# Autodesk Inventor assembly: Chimera Assembly
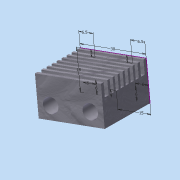
[picture p0: Inventor's stored thumbnail of the model, 180x180]
Saved by Autodesk Inventor 2016 (Build 200138000, 138)
## iProperties
Created: 2016-08-02
Part Number: Chimera Assembly
Document SubType Name: Assembly
Designer: Sam
Author: Sam
## Documents named in this file (3)
- D:\Users\Sam\Documents\Inventor\Zircon3D\Chimera Assembly.iam
- D:\Users\Sam\Documents\Inventor\Zircon3D\Chimera Heatsink.ipt
- D:\Users\Sam\Documents\Inventor\Zircon3D\Chimera Hetsink Brass Insert.ipt
## Components (3 placed, 2 different names)
1. Chimera Heatsink:1 — Rotational:1, Rotational:2
2. Chimera Hetsink Brass Insert:1 — Rotational:1
3. Chimera Hetsink Brass Insert:2 — Rotational:2
## Relationships (2: RevoluteJoint 2)
- Rotational:1 [RevoluteJoint]: Chimera Heatsink:1 ↔ Chimera Hetsink Brass Insert:1
- Rotational:2 [RevoluteJoint]: Chimera Heatsink:1 ↔ Chimera Hetsink Brass Insert:2
